# Autodesk Inventor assembly: hindge
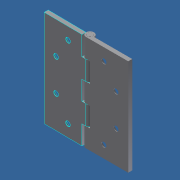
[picture p0: Inventor's stored thumbnail of the model, 180x180]
Saved by Autodesk Inventor 2011 SP1 (Build 150282100, 282)
## iProperties
Created: 2011-06-12
Part Number: hindge
Document SubType Name: Assembly
Designer: john
Author: john
## Documents named in this file (4)
- C:\Documents and Settings\john\My Documents\Inventor\ProjectName\hindge.iam
- C:\Documents and Settings\john\My Documents\Inventor\ProjectName\hindge 1.ipt
- C:\Documents and Settings\john\My Documents\Inventor\ProjectName\Part2.ipt
- C:\Documents and Settings\john\My Documents\Inventor\ProjectName\pin.ipt
## Components (3 placed, 3 different names)
1. hindge 1:1 — Mate:1, Flush:1, Flush:2
2. Part2:1 — Mate:1, Flush:1
3. pin:1 — Flush:2
## Relationships (3: Flush 2, Mate 1)
- Mate:1: hindge 1:1 ↔ Part2:1
- Flush:1: hindge 1:1 ↔ Part2:1
- Flush:2: hindge 1:1 ↔ pin:1
